# Autodesk Inventor assembly: Chassi 12-16-2019
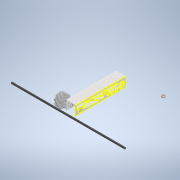
[picture p0: Inventor's stored thumbnail of the model, 180x180]
Saved by Autodesk Inventor 2021 (Build 250183000, 183)
## iProperties
Created: 2019-12-09
Part Number: Chassi 12-16-2019
Document SubType Name: Assembly
Designer: deli
Author: deli
## Documents named in this file (11)
- C:\Users\deli\OneDrive - Eastside Preparatory School\FTC\Chassi\Chassi 12-16-2019.iam
- C:\Users\deli\OneDrive - Eastside Preparatory School\FTC\Chassi\38007_txm-aluminum bevel gearing.ipt
- C:\Users\deli\OneDrive - Eastside Preparatory School\FTC\Chassi\am-3215 6mm D bore Double Nub.ipt
- C:\Users\deli\OneDrive - Eastside Preparatory School\FTC\Chassi\am-3637 NeveRest Orbital 20 Gearmotor REV2.ipt
- C:\Users\deli\OneDrive - Eastside Preparatory School\FTC\Chassi\Side Channel.ipt
- C:\Users\deli\OneDrive - Eastside Preparatory School\FTC\Chassi\_32t_Aluminum_Plate_Sprocket_25_Chain_1-1_8_Bearing_Bore_217-2690.ipt
- C:\Users\deli\OneDrive - Eastside Preparatory School\FTC\Chassi\1_2_Hex_x_0_201_ID_ThunderHex_Stock_36_217-4017.ipt
- C:\Users\deli\OneDrive - Eastside Preparatory School\FTC\Chassi\100 mm mecanum wheel.ipt
- C:\Users\deli\OneDrive - Eastside Preparatory School\FTC\Chassi\0_500_Hex_ID_x_1_125_OD_x_0_313_WD_Flanged_Bearing_v2_217-3875 v1.ipt
- C:\Users\deli\OneDrive - Eastside Preparatory School\FTC\Chassi\MecanumSideplates v1.ipt
- C:\Users\deli\OneDrive - Eastside Preparatory School\FTC\Chassi\MecanumSideplatesShort v1.ipt
## Components (20 placed, 10 different names)
1. 38007_txm-aluminum bevel gearing:1
2. am-3215 6mm D bore Double Nub:1
3. am-3637 NeveRest Orbital 20 Gearmotor REV2:1
4. 38007_txm-aluminum bevel gearing:2 — Mate:4, Mate:5
5. am-3215 6mm D bore Double Nub:2 — Mate:1, Mate:2, Mate:3, Mate:4, Mate:5
6. am-3637 NeveRest Orbital 20 Gearmotor REV2:2 — Mate:1, Mate:2, Mate:3
7. 38007_txm-aluminum bevel gearing:3
8. am-3215 6mm D bore Double Nub:3
9. am-3637 NeveRest Orbital 20 Gearmotor REV2:3
10. 38007_txm-aluminum bevel gearing:4
11. am-3215 6mm D bore Double Nub:4
12. am-3637 NeveRest Orbital 20 Gearmotor REV2:4
13. Side Channel:1 — Mate:17, Mate:18
14. _32t_Aluminum_Plate_Sprocket_25_Chain_1-1_8_Bearing_Bore_217-2690:1 — Mate:6, Mate:15
15. 1_2_Hex_x_0_201_ID_ThunderHex_Stock_36_217-4017:1 — Mate:16, Angle:2
16. 100 mm mecanum wheel:1 — Mate:6, Mate:8, Mate:9, Mate:10, Mate:11, Mate:12, Mate:13, Mate:14
17. 0_500_Hex_ID_x_1_125_OD_x_0_313_WD_Flanged_Bearing_v2_217-3875 v1:1 — Mate:8, Angle:1, Mate:17, Mate:18
18. 0_500_Hex_ID_x_1_125_OD_x_0_313_WD_Flanged_Bearing_v2_217-3875 v1:2
19. MecanumSideplates v1:1 — Mate:12, Mate:13, Mate:14
20. MecanumSideplatesShort v1:1 — Mate:9, Mate:10, Mate:11, Mate:15, Angle:1, Mate:16, Angle:2
## Relationships (19: Mate 17, Angle 2)
- Mate:1: am-3215 6mm D bore Double Nub:2 ↔ am-3637 NeveRest Orbital 20 Gearmotor REV2:2
- Mate:2: am-3215 6mm D bore Double Nub:2 ↔ am-3637 NeveRest Orbital 20 Gearmotor REV2:2
- Mate:3: am-3215 6mm D bore Double Nub:2 ↔ am-3637 NeveRest Orbital 20 Gearmotor REV2:2
- Mate:4: 38007_txm-aluminum bevel gearing:2 ↔ am-3215 6mm D bore Double Nub:2
- Mate:5: 38007_txm-aluminum bevel gearing:2 ↔ am-3215 6mm D bore Double Nub:2
- Mate:6: _32t_Aluminum_Plate_Sprocket_25_Chain_1-1_8_Bearing_Bore_217-2690:1 ↔ 100 mm mecanum wheel:1
- Mate:8: 100 mm mecanum wheel:1 ↔ 0_500_Hex_ID_x_1_125_OD_x_0_313_WD_Flanged_Bearing_v2_217-3875 v1:1
- Mate:9: 100 mm mecanum wheel:1 ↔ MecanumSideplatesShort v1:1
- Mate:10: 100 mm mecanum wheel:1 ↔ MecanumSideplatesShort v1:1
- Mate:11: 100 mm mecanum wheel:1 ↔ MecanumSideplatesShort v1:1
- Mate:12: 100 mm mecanum wheel:1 ↔ MecanumSideplates v1:1
- Mate:13: 100 mm mecanum wheel:1 ↔ MecanumSideplates v1:1
- Mate:14: 100 mm mecanum wheel:1 ↔ MecanumSideplates v1:1
- Mate:15: _32t_Aluminum_Plate_Sprocket_25_Chain_1-1_8_Bearing_Bore_217-2690:1 ↔ MecanumSideplatesShort v1:1
- Angle:1 (0 deg): 0_500_Hex_ID_x_1_125_OD_x_0_313_WD_Flanged_Bearing_v2_217-3875 v1:1 ↔ MecanumSideplatesShort v1:1
- Mate:16: 1_2_Hex_x_0_201_ID_ThunderHex_Stock_36_217-4017:1 ↔ MecanumSideplatesShort v1:1
- Angle:2 (0 deg): 1_2_Hex_x_0_201_ID_ThunderHex_Stock_36_217-4017:1 ↔ MecanumSideplatesShort v1:1
- Mate:17: Side Channel:1 ↔ 0_500_Hex_ID_x_1_125_OD_x_0_313_WD_Flanged_Bearing_v2_217-3875 v1:1
- Mate:18: Side Channel:1 ↔ 0_500_Hex_ID_x_1_125_OD_x_0_313_WD_Flanged_Bearing_v2_217-3875 v1:1
